# Autodesk Inventor assembly: Ball Collection Mechanism
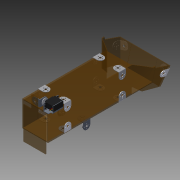
[picture p0: Inventor's stored thumbnail of the model, 180x180]
Saved by Autodesk Inventor 2015 SP1 (Build 190203100, 203)
## iProperties
Created: 2014-09-14
Part Number: Ball Collection Mechanism
Document SubType Name: Assembly
Designer: Family Room
Author: Family Room
## Documents named in this file (9)
- C:\Users\datenney\Documents\GitHub\CAD\2014_robotComplete\Ball Collection Mechanism.iam
- C:\Users\datenney\Documents\GitHub\CAD\2014_robotComplete\Imported Components\L bracket\L bracket.ipt
- C:\Users\datenney\Documents\GitHub\CAD\2014_robotComplete\Ball Collector.ipt
- C:\Users\datenney\Documents\GitHub\CAD\2014_robotComplete\Imported Components\Motor Hub\Motor Hub.ipt
- C:\Users\datenney\Documents\GitHub\CAD\2014_robotComplete\Imported Components\40 tooth Gear\40 tooth Gear.ipt
- C:\Users\datenney\Documents\GitHub\CAD\2014_robotComplete\Imported Components\singleservobracket\singleservobracket.ipt
- C:\Users\datenney\Documents\GitHub\CAD\2014_robotComplete\Imported Components\servo\servo.iam
- C:\Users\datenney\Documents\GitHub\CAD\2014_robotComplete\Ball Release.ipt
- C:\Users\datenney\Documents\GitHub\CAD\COTSParts\Tetrix\Tetrix bracket - angle.ipt
## Components (20 placed, 8 different names)
1. L bracket:1 — Mate:2, Flush:2, Flush:3, Insert:5, Insert:6, Flush:8
2. L bracket:2 — Mate:1, Flush:1, Flush:3, Insert:1
3. Ball Collector:1 — Mate:1, Flush:1, Mate:2, Flush:2, Mate:5, Flush:5, Flush:7, Flush:8, Mate:10, Mate:11, Mate:14, Mate:15, Mate:17, Mate:18, Mate:19, Mate:20, Mate:21, Mate:22, Mate:24, Mate:26, Mate:27, Mate:30, Mate:31, Mate:32, Mate:33, Mate:34, Mate:35, Mate:36
4. Motor Hub:1 — Insert:5
5. Motor Hub:2 — Insert:1
6. 40 tooth Gear:1 — Insert:6
7. singleservobracket:1 — Mate:3, Angle:1, Mate:4, Mate:5, Flush:7
8. servo:1 [sub-assembly] — Mate:3, Angle:1, Mate:4, Insert:4
9. L bracket:3 — Insert:4, Flush:5, Mate:6, Mate:7, Mate:8
10. Ball Release:1 — Mate:6, Mate:7, Mate:8
11. Tetrix bracket - angle:1 — Mate:10, Mate:21
12. Tetrix bracket - angle:2 — Mate:11, Mate:22
13. Tetrix bracket - angle:3 — Mate:15, Mate:20
14. Tetrix bracket - angle:4 — Mate:14, Mate:17
15. Tetrix bracket - angle:6 — Mate:27, Mate:32, Mate:33
16. Tetrix bracket - angle:7 — Mate:30, Mate:31
17. Tetrix bracket - angle:8 — Mate:26
18. Tetrix bracket - angle:9 — Mate:24
19. Tetrix bracket - angle:10 — Mate:18, Mate:19
20. Tetrix bracket - angle:11 — Mate:34, Mate:35, Mate:36
## Relationships (39: Mate 28, Flush 6, Insert 4, Angle 1)
- Mate:1: L bracket:2 ↔ Ball Collector:1
- Flush:1: L bracket:2 ↔ Ball Collector:1
- Mate:2: L bracket:1 ↔ Ball Collector:1
- Flush:2: L bracket:1 ↔ Ball Collector:1
- Flush:3: L bracket:1 ↔ L bracket:2
- Insert:1: L bracket:2 ↔ Motor Hub:2
- Mate:3: singleservobracket:1 ↔ servo:1
- Angle:1 (0 deg): singleservobracket:1 ↔ servo:1
- Mate:4: singleservobracket:1 ↔ servo:1
- Insert:4: servo:1 ↔ L bracket:3
- Mate:5: Ball Collector:1 ↔ singleservobracket:1
- Flush:5: Ball Collector:1 ↔ L bracket:3
- Mate:6: L bracket:3 ↔ Ball Release:1
- Mate:7: L bracket:3 ↔ Ball Release:1
- Mate:8: L bracket:3 ↔ Ball Release:1
- Flush:7 (-2.286 mm): Ball Collector:1 ↔ singleservobracket:1
- Insert:5: L bracket:1 ↔ Motor Hub:1
- Insert:6: L bracket:1 ↔ 40 tooth Gear:1
- Flush:8 (139.7 mm): L bracket:1 ↔ Ball Collector:1
- Mate:10: Ball Collector:1 ↔ Tetrix bracket - angle:1
- Mate:11: Ball Collector:1 ↔ Tetrix bracket - angle:2
- Mate:14: Ball Collector:1 ↔ Tetrix bracket - angle:4
- Mate:15: Ball Collector:1 ↔ Tetrix bracket - angle:3
- Mate:17: Ball Collector:1 ↔ Tetrix bracket - angle:4
- Mate:18: Ball Collector:1 ↔ Tetrix bracket - angle:10
- Mate:19: Ball Collector:1 ↔ Tetrix bracket - angle:10
- Mate:20: Ball Collector:1 ↔ Tetrix bracket - angle:3
- Mate:21: Ball Collector:1 ↔ Tetrix bracket - angle:1
- Mate:22: Ball Collector:1 ↔ Tetrix bracket - angle:2
- Mate:24: Ball Collector:1 ↔ Tetrix bracket - angle:9
- Mate:26: Ball Collector:1 ↔ Tetrix bracket - angle:8
- Mate:27: Ball Collector:1 ↔ Tetrix bracket - angle:6
- Mate:30: Ball Collector:1 ↔ Tetrix bracket - angle:7
- Mate:31: Ball Collector:1 ↔ Tetrix bracket - angle:7
- Mate:32: Ball Collector:1 ↔ Tetrix bracket - angle:6
- Mate:33: Ball Collector:1 ↔ Tetrix bracket - angle:6
- Mate:34: Ball Collector:1 ↔ Tetrix bracket - angle:11
- Mate:35: Ball Collector:1 ↔ Tetrix bracket - angle:11
- Mate:36: Ball Collector:1 ↔ Tetrix bracket - angle:11
